# Autodesk Inventor assembly: claw_static_gripper_assembly
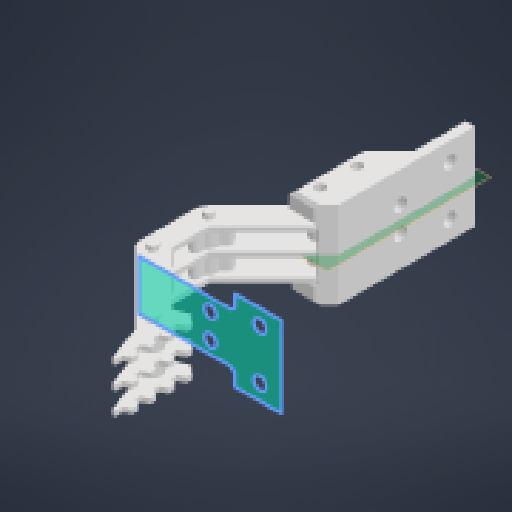
[picture p0: Inventor's stored thumbnail of the model, 512x512]
Saved by Autodesk Inventor 2026 (Build 300175000, 175)
## iProperties
Created: 2025-03-27
Part Number: claw_static_gripper_assembly
Document SubType Name: Assembly
Designer: paris
Author: paris
## Documents named in this file (7)
- C:\Users\paris\OneDrive\Desktop\claw_manipulator_designs_final\claw_static_gripper_assembly.iam
- C:\Users\paris\OneDrive\Desktop\claw_manipulator_designs_final\claw_gripper.ipt
- C:\Users\paris\OneDrive\Desktop\claw_manipulator_designs_final\claw_connecting_rod.ipt
- C:\Users\paris\OneDrive\Desktop\claw_manipulator_designs_final\claw_joined_spacer.ipt
- C:\Users\paris\OneDrive\Desktop\claw_manipulator_designs_final\claw_spacer.ipt
- C:\Users\paris\OneDrive\Desktop\claw_manipulator_designs_final\claw_static_mount.ipt
- C:\Users\paris\OneDrive\Desktop\claw_manipulator_designs_final\claw_static_mount_rod.ipt
## Components (20 placed, 7 different names)
1. claw_gripper:1 — Flush:1, Mate:1, Mate:2, Mate:3, Mate:4, Flush:2, Mate:6, Angle:1, Flush:3, Mate:7, Mate:8, Mate:9, Mate:10, Mate:27, Mate:28, Flush:4, Flush:5
2. claw_connecting_rod:1 — Flush:1, Mate:12, Mate:14, Mate:24
3. claw_connecting_rod:2 — Mate:1, Mate:2, Mate:5, Mate:11, Mate:15, Mate:25
4. claw_connecting_rod:3 — Mate:3, Mate:4, Mate:16
5. claw_gripper:2 — Mate:11, Mate:12, Mate:13, Mate:17, Mate:18, Mate:19, Mate:20, Mate:21, Mate:22, Mate:23, Angle:2, Angle:3
6. claw_angled_spacer — Flush:2
7. claw_joined_spacer:2 — Mate:5, Mate:6, Angle:1, Mate:13
8. claw_spacer:1 — Flush:3
9. claw_spacer:2 — Mate:7, Mate:8
10. claw_spacer:3 — Mate:9, Mate:10
11. claw_joined_spacer:3 — Mate:14, Mate:19, Angle:3
12. claw_joined_spacer:4 — Mate:15, Mate:20, Angle:2, Mate:26
13. claw_spacer:4 — Mate:16, Mate:23
14. claw_spacer:5 — Mate:17, Mate:21
15. claw_spacer:6 — Mate:18, Mate:22
16. claw_gripper:3 — Mate:24, Mate:25, Mate:26, Flush:6
17. claw_connecting_rod:4 — Mate:28, Flush:5
18. claw_connecting_rod:5 — Mate:27, Flush:4
19. claw_static_mount:1 — Flush:6, Flush:7
20. claw_static_mount_rod:1 — Flush:7
## Relationships (38: Mate 28, Flush 7, Angle 3)
- Flush:1 (2 mm): claw_gripper:1 ↔ claw_connecting_rod:1
- Mate:1: claw_gripper:1 ↔ claw_connecting_rod:2
- Mate:2 (2 mm): claw_gripper:1 ↔ claw_connecting_rod:2
- Mate:3: claw_gripper:1 ↔ claw_connecting_rod:3
- Mate:4 (2 mm): claw_gripper:1 ↔ claw_connecting_rod:3
- Flush:2: claw_gripper:1 ↔ claw_angled_spacer
- Mate:5: claw_connecting_rod:2 ↔ claw_joined_spacer:2
- Mate:6: claw_gripper:1 ↔ claw_joined_spacer:2
- Angle:1 (0 deg): claw_gripper:1 ↔ claw_joined_spacer:2
- Flush:3: claw_gripper:1 ↔ claw_spacer:1
- Mate:7: claw_gripper:1 ↔ claw_spacer:2
- Mate:8: claw_gripper:1 ↔ claw_spacer:2
- Mate:9: claw_gripper:1 ↔ claw_spacer:3
- Mate:10: claw_gripper:1 ↔ claw_spacer:3
- Mate:11: claw_connecting_rod:2 ↔ claw_gripper:2
- Mate:12: claw_connecting_rod:1 ↔ claw_gripper:2
- Mate:13: claw_gripper:2 ↔ claw_joined_spacer:2
- Mate:14: claw_connecting_rod:1 ↔ claw_joined_spacer:3
- Mate:15: claw_connecting_rod:2 ↔ claw_joined_spacer:4
- Mate:16: claw_connecting_rod:3 ↔ claw_spacer:4
- Mate:17: claw_gripper:2 ↔ claw_spacer:5
- Mate:18: claw_gripper:2 ↔ claw_spacer:6
- Mate:19: claw_gripper:2 ↔ claw_joined_spacer:3
- Mate:20: claw_gripper:2 ↔ claw_joined_spacer:4
- Mate:21: claw_gripper:2 ↔ claw_spacer:5
- Mate:22: claw_gripper:2 ↔ claw_spacer:6
- Mate:23: claw_gripper:2 ↔ claw_spacer:4
- Angle:2 (0 deg): claw_gripper:2 ↔ claw_joined_spacer:4
- Angle:3 (0 deg): claw_gripper:2 ↔ claw_joined_spacer:3
- Mate:24: claw_connecting_rod:1 ↔ claw_gripper:3
- Mate:25: claw_connecting_rod:2 ↔ claw_gripper:3
- Mate:26: claw_joined_spacer:4 ↔ claw_gripper:3
- Mate:27: claw_gripper:1 ↔ claw_connecting_rod:5
- Mate:28: claw_gripper:1 ↔ claw_connecting_rod:4
- Flush:4 (-2 mm): claw_gripper:1 ↔ claw_connecting_rod:5
- Flush:5 (-2 mm): claw_gripper:1 ↔ claw_connecting_rod:4
- Flush:6: claw_gripper:3 ↔ claw_static_mount:1
- Flush:7: claw_static_mount:1 ↔ claw_static_mount_rod:1
